# Autodesk Inventor assembly: Băng chuyền
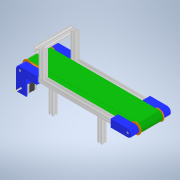
[picture p0: Inventor's stored thumbnail of the model, 180x180]
Saved by Autodesk Inventor 2020 (Build 240168000, 168)
## iProperties
_SolveAssemblyDoc: Frame Generator Solve Assembly
_Version: 15.0.0
Created: 2022-11-30
Part Number: Băng chuyền
Document SubType Name: Assembly
Designer: ADMIN
Author: ADMIN
## Documents named in this file (9)
- D:\Do-an-tot-nghiep\Inventor\Băng chuyền.iam
- D:\Do-an-tot-nghiep\Inventor\băng chuyền.ipt
- D:\Do-an-tot-nghiep\Inventor\bangchuyenstep.ipt
- D:\Do-an-tot-nghiep\Inventor\truc_bang_chuyen.ipt
- C:\Users\ADMIN\OneDrive\Documents\Inventor\Content Center Files\R2020\en-US\ISO 2338(2)\ISO 2338 - 8 h8 x 120.ipt
- C:\Users\ADMIN\OneDrive\Documents\Khung nhôm băng chuyền.ipt
- D:\Do-an-tot-nghiep\Inventor\step\Assembly1.iam
- D:\Do-an-tot-nghiep\Inventor\Băng chuyền\Frame\Frame 1670595420372.iam
- D:\Do-an-tot-nghiep\Inventor\Băng tải.ipt
## Components (12 placed, 8 different names)
1. băng chuyền:1 — Flush:2, Flush:3, Flush:4, Mate:8, Mate:13, Flush:5, Mate:27
2. bangchuyenstep:1 — Flush:3, Mate:7, Mate:10, Flush:5, Mate:21, Mate:22, Flush:6, Mate:23, Flush:7, Flush:8, Flush:9
3. băng chuyền:2 — Flush:2, Mate:2, Flush:4, Mate:9, Mate:12, Mate:25, Mate:26
4. băng chuyền:3 — Mate:2, Mate:6, Mate:11, Mate:24, Flush:10
5. truc_bang_chuyen:1 — Mate:6, Mate:9, Mate:11
6. truc_bang_chuyen:2 — Mate:7, Mate:8, Mate:10
7. ISO 2338 8 h8 x 120:1 — Mate:12, Flush:10
8. ISO 2338 8 h8 x 120:2 — Mate:13, Flush:9
9. Khung nhôm băng chuyền:1
10. Assembly1:1 [sub-assembly] — Mate:21, Mate:22, Flush:6
11. Frame 1670595420372:1 [sub-assembly] — Mate:23, Flush:7, Flush:8, Mate:24
12. Băng tải:1 — Mate:25, Mate:26, Mate:27
## Relationships (25: Mate 16, Flush 9)
- Flush:2: băng chuyền:1 ↔ băng chuyền:2
- Flush:3: băng chuyền:1 ↔ bangchuyenstep:1
- Mate:2: băng chuyền:2 ↔ băng chuyền:3
- Flush:4: băng chuyền:1 ↔ băng chuyền:2
- Mate:6: băng chuyền:3 ↔ truc_bang_chuyen:1
- Mate:7: bangchuyenstep:1 ↔ truc_bang_chuyen:2
- Mate:8 (1 mm): băng chuyền:1 ↔ truc_bang_chuyen:2
- Mate:9 (1 mm): băng chuyền:2 ↔ truc_bang_chuyen:1
- Mate:10 (1 mm): bangchuyenstep:1 ↔ truc_bang_chuyen:2
- Mate:11 (1 mm): băng chuyền:3 ↔ truc_bang_chuyen:1
- Mate:12: băng chuyền:2 ↔ ISO 2338 8 h8 x 120:1
- Mate:13: băng chuyền:1 ↔ ISO 2338 8 h8 x 120:2
- Flush:5: băng chuyền:1 ↔ bangchuyenstep:1
- Mate:21: bangchuyenstep:1 ↔ Assembly1:1
- Mate:22: bangchuyenstep:1 ↔ Assembly1:1
- Flush:6: bangchuyenstep:1 ↔ Assembly1:1
- Mate:23: bangchuyenstep:1 ↔ Frame 1670595420372:1
- Flush:7 (20 mm): bangchuyenstep:1 ↔ Frame 1670595420372:1
- Flush:8 (-20 mm): bangchuyenstep:1 ↔ Frame 1670595420372:1
- Mate:24: băng chuyền:3 ↔ Frame 1670595420372:1
- Flush:9: bangchuyenstep:1 ↔ ISO 2338 8 h8 x 120:2
- Flush:10: băng chuyền:3 ↔ ISO 2338 8 h8 x 120:1
- Mate:25: băng chuyền:2 ↔ Băng tải:1
- Mate:26 (4 mm): băng chuyền:2 ↔ Băng tải:1
- Mate:27: băng chuyền:1 ↔ Băng tải:1
